# Autodesk Inventor assembly: 回路全部2
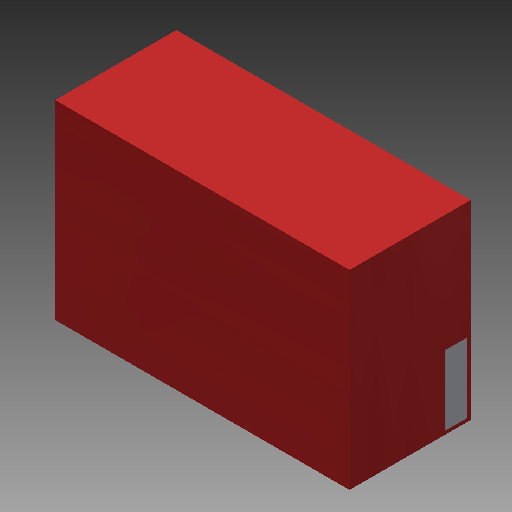
[picture p0: Inventor's stored thumbnail of the model, 512x512]
Saved by Autodesk Inventor 2020 (Build 240168000, 168)
## iProperties
Created: 2018-11-30
Part Number: 回路全部2
Material: 一般
Document SubType Name: Assembly
Designer: 雪村
Mass: 142 g
Surface Area: 315.438 cm^2
Volume: 191.977 cm^3
Density: 0.739671 g/cm^3
Author: 雪村
## Documents named in this file (5)
- C:\Users\white\Documents\SRDC\SRDC\Inventor_2017\2018年機体\パーツ\回路全部2.iam
- C:\Users\white\Documents\SRDC\SRDC\Inventor_2017\2018年機体\パーツ\回路2.ipt
- C:\Users\white\Documents\SRDC\SRDC\Inventor_2017\2018年機体\パーツ\MC402CR.ipt
- C:\Users\white\Documents\SRDC\SRDC\Inventor_2017\2018年機体\パーツ\サイドワインダーマイクロ2.ipt
- C:\Users\white\Documents\SRDC\SRDC\Inventor_2017\2018年機体\パーツ\受信機.ipt
## Components (5 placed, 4 different names)
1. 回路2:1 — フラッシュ:1, フラッシュ:2, フラッシュ:3, フラッシュ:4, フラッシュ:5, フラッシュ:6, フラッシュ:7
2. MC402CR:1 — フラッシュ:4, メイト:3, メイト:4
3. サイドワインダーマイクロ2:1 — フラッシュ:3, メイト:2, フラッシュ:8, メイト:3
4. 受信機:1 — フラッシュ:1, フラッシュ:5, フラッシュ:6, メイト:1, メイト:4
5. サイドワインダーマイクロ2:2 — フラッシュ:2, フラッシュ:7, メイト:1, メイト:2, フラッシュ:8
## Relationships (12: Flush 8, Mate 4)
- フラッシュ:1 [Flush]: 回路2:1 ↔ 受信機:1
- フラッシュ:2 [Flush]: 回路2:1 ↔ サイドワインダーマイクロ2:2
- フラッシュ:3 [Flush]: 回路2:1 ↔ サイドワインダーマイクロ2:1
- フラッシュ:4 [Flush]: 回路2:1 ↔ MC402CR:1
- フラッシュ:5 [Flush]: 回路2:1 ↔ 受信機:1
- フラッシュ:6 [Flush]: 回路2:1 ↔ 受信機:1
- フラッシュ:7 [Flush]: 回路2:1 ↔ サイドワインダーマイクロ2:2
- メイト:1 [Mate]: 受信機:1 ↔ サイドワインダーマイクロ2:2
- メイト:2 [Mate]: サイドワインダーマイクロ2:1 ↔ サイドワインダーマイクロ2:2
- フラッシュ:8 [Flush]: サイドワインダーマイクロ2:1 ↔ サイドワインダーマイクロ2:2
- メイト:3 [Mate]: MC402CR:1 ↔ サイドワインダーマイクロ2:1
- メイト:4 [Mate]: MC402CR:1 ↔ 受信機:1
